# Autodesk Inventor assembly: bat_pack
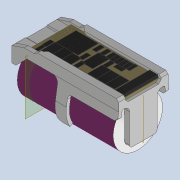
[picture p0: Inventor's stored thumbnail of the model, 180x180]
Saved by Autodesk Inventor 2020 (Build 240168000, 168)
## iProperties
Created: 2021-08-25
Part Number: bat_pack
Document SubType Name: Assembly
Designer: Shuang Peng
Author: Shuang Peng
## Documents named in this file (4)
- D:\projects-3\soft module robot\hardware\diff module 3\bat_pack.iam
- D:\projects-3\soft module robot\hardware\diff module 3\ele\dc_dc_2 v1\dc_dc_2.iam
- D:\projects-3\soft module robot\hardware\diff module 3\bat_18350.ipt
- D:\projects-3\soft module robot\hardware\diff module 3\bat_pack_1.ipt
## Components (3 placed, 3 different names)
1. dc_dc_2:1 [sub-assembly] — Flush:2, Tangent:3, Tangent:4, Flush:3, Mate:2, Mate:3
2. bat_18350:1 — Flush:2, Tangent:3, Tangent:4
3. bat_pack_1:1 — Flush:3, Mate:2, Mate:3
## Relationships (6: Flush 2, Tangent 2, Mate 2)
- Flush:2 (1 mm): dc_dc_2:1 ↔ bat_18350:1
- Tangent:3 (1 mm): dc_dc_2:1 ↔ bat_18350:1
- Tangent:4 (-1.5 mm): dc_dc_2:1 ↔ bat_18350:1
- Flush:3: dc_dc_2:1 ↔ bat_pack_1:1
- Mate:2: dc_dc_2:1 ↔ bat_pack_1:1
- Mate:3: dc_dc_2:1 ↔ bat_pack_1:1
